# Autodesk Inventor assembly: Baugruppe1
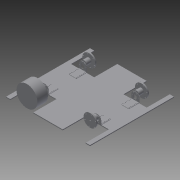
[picture p0: Inventor's stored thumbnail of the model, 180x180]
Saved by Autodesk Inventor 2014 (Build 180170000, 170)
## iProperties
Created: 2015-10-03
Part Number: Baugruppe1
Document SubType Name: Assembly
Designer: Home
Author: Home
## Documents named in this file (5)
- C:\Users\nrk\git\raw.bot\misc\Baugruppe1.iam
- C:\Users\nrk\git\raw.bot\misc\Motorhalterung.ipt
- C:\Users\nrk\git\raw.bot\misc\Bodenplatte.ipt
- C:\Users\nrk\git\raw.bot\misc\6 mm Set Hub.ipt
- C:\Users\nrk\git\raw.bot\misc\Rad.ipt
## Components (10 placed, 4 different names)
1. Motorhalterung:1 — Starr:4, Drehbar:3
2. Motorhalterung:2 — Starr:2, Drehbar:4
3. Motorhalterung:3 — Starr:3, Drehbar:1
4. Motorhalterung:4 — Starr:1, Drehbar:2
5. Bodenplatte:1 — Starr:1, Starr:2, Starr:3, Starr:4
6. 6 mm Set Hub:1 — Drehbar:2
7. 6 mm Set Hub:2 — Drehbar:1
8. 6 mm Set Hub:3 — Drehbar:3, Drehbar:5
9. 6 mm Set Hub:4 — Drehbar:4
10. Rad:1 — Drehbar:5
## Relationships (9: RevoluteJoint 5, WeldJoint 4)
- Starr:1 [WeldJoint]: Motorhalterung:4 ↔ Bodenplatte:1
- Starr:2 [WeldJoint]: Motorhalterung:2 ↔ Bodenplatte:1
- Starr:3 [WeldJoint]: Motorhalterung:3 ↔ Bodenplatte:1
- Starr:4 [WeldJoint]: Motorhalterung:1 ↔ Bodenplatte:1
- Drehbar:1 [RevoluteJoint] (6 mm): Motorhalterung:3 ↔ 6 mm Set Hub:2
- Drehbar:2 [RevoluteJoint] (6 mm): Motorhalterung:4 ↔ 6 mm Set Hub:1
- Drehbar:3 [RevoluteJoint] (6 mm): Motorhalterung:1 ↔ 6 mm Set Hub:3
- Drehbar:4 [RevoluteJoint] (6 mm): Motorhalterung:2 ↔ 6 mm Set Hub:4
- Drehbar:5 [RevoluteJoint]: 6 mm Set Hub:3 ↔ Rad:1
